# Autodesk Inventor assembly: high_joint
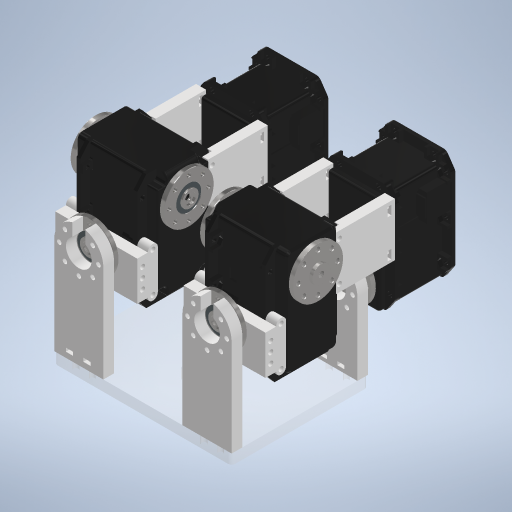
[picture p0: Inventor's stored thumbnail of the model, 512x512]
Saved by Autodesk Inventor 2024.3 (Build 283343000, 343)
## iProperties
Created: 2024-09-16
Part Number: high_joint
Document SubType Name: Assembly
Designer: USER
Author: USER
## Documents named in this file (10)
- C:\Users\USER\Desktop\로빛 예비인턴\(git)19기 이원준 격투로봇 설계파일\Lower_body\high_joint.iam
- C:\Users\USER\Desktop\로빛 예비인턴\(git)19기 이원준 격투로봇 설계파일\Lower_body\_pelvis.ipt
- C:\Users\USER\Desktop\로빛 예비인턴\(git)19기 이원준 격투로봇 설계파일\Lower_body\_thigh_adt_body.ipt
- C:\Users\USER\Desktop\로빛 예비인턴\(git)19기 이원준 격투로봇 설계파일\Lower_body\_foot_adt.ipt
- C:\Users\USER\Desktop\로빛 예비인턴\(git)19기 이원준 격투로봇 설계파일\Lower_body\_idle_adt.ipt
- C:\Users\USER\Desktop\로빛 예비인턴\(git)19기 이원준 격투로봇 설계파일\Lower_body\_adle_adt_2.ipt
- C:\Users\USER\Desktop\로빛 예비인턴\(git)19기 이원준 격투로봇 설계파일\아이들러\64아이들러.iam
- C:\Users\USER\Desktop\로빛 예비인턴\(git)19기 이원준 격투로봇 설계파일\motor\Motor_64_no_idle_ver.iam
- C:\Users\USER\Desktop\로빛 예비인턴\(git)19기 이원준 격투로봇 설계파일\motor\Motor_106.iam
- C:\Users\USER\Desktop\로빛 예비인턴\(git)19기 이원준 격투로봇 설계파일\Lower_body\_108-64_adt.ipt
## Components (21 placed, 9 different names)
1. _pelvis:1 — 플러쉬:1, 플러쉬:2, 삽입:1, 삽입:2, 각도:4, 삽입:3, 삽입:4, 각도:5, 각도:8, 삽입:5, 삽입:6, 삽입:7, 삽입:8
2. _thigh_adt_body:3 — 삽입:1, 삽입:2, 각도:7, 삽입:24, 각도:11, 각도:12, 삽입:38
3. _thigh_adt_body:4 — 각도:4, 삽입:3, 삽입:4, 각도:6, 삽입:23, 각도:10, 각도:13, 삽입:39
4. _foot_adt:1 — 각도:5, 각도:6, 삽입:5, 삽입:6, 삽입:25
5. _foot_adt:2 — 각도:7, 각도:8, 삽입:7, 삽입:8, 삽입:26
6. _idle_adt:3
7. _idle_adt:4 — 삽입:29, 삽입:30
8. _adle_adt_2:2 — 삽입:17
9. 64아이들러:1 [sub-assembly] — 삽입:17, 삽입:24, 삽입:38
10. _idle_adt:5 — 삽입:27, 삽입:28
11. _idle_adt:6
12. _adle_adt_2:3
13. 64아이들러:2 [sub-assembly] — 삽입:23, 삽입:39
14. Motor_64_no_idle_ver:1 [sub-assembly] — 삽입:26, 삽입:35, 삽입:36, 삽입:37, 각도:16
15. Motor_64_no_idle_ver:2 [sub-assembly] — 삽입:25, 삽입:31, 삽입:32, 삽입:33, 삽입:34
16. Motor_106:1 [sub-assembly] — 각도:11, 각도:12, 삽입:29, 삽입:30, 각도:16
17. Motor_106:2 [sub-assembly] — 각도:10, 각도:13, 삽입:27, 삽입:28, 각도:15
18. _108-64_adt:1 — 각도:14, 삽입:35, 삽입:36
19. _108-64_adt:2 — 각도:14, 삽입:37
20. _108-64_adt:3 — 삽입:33, 삽입:34
21. _108-64_adt:4 — 삽입:31, 삽입:32, 각도:15
## Relationships (49: Insert 35, Angle 12, Flush 2)
- 플러쉬:1 [Flush]: _pelvis:1
- 플러쉬:2 [Flush]: _pelvis:1
- 삽입:1 [Insert]: _pelvis:1 ↔ _thigh_adt_body:3
- 삽입:2 [Insert]: _pelvis:1 ↔ _thigh_adt_body:3
- 각도:4 [Angle] (0 deg): _pelvis:1 ↔ _thigh_adt_body:4
- 삽입:3 [Insert]: _pelvis:1 ↔ _thigh_adt_body:4
- 삽입:4 [Insert]: _pelvis:1 ↔ _thigh_adt_body:4
- 각도:5 [Angle] (0 deg): _pelvis:1 ↔ _foot_adt:1
- 각도:6 [Angle] (0 deg): _thigh_adt_body:4 ↔ _foot_adt:1
- 각도:7 [Angle] (0 deg): _thigh_adt_body:3 ↔ _foot_adt:2
- 각도:8 [Angle] (0 deg): _pelvis:1 ↔ _foot_adt:2
- 삽입:5 [Insert]: _pelvis:1 ↔ _foot_adt:1
- 삽입:6 [Insert]: _pelvis:1 ↔ _foot_adt:1
- 삽입:7 [Insert]: _pelvis:1 ↔ _foot_adt:2
- 삽입:8 [Insert]: _pelvis:1 ↔ _foot_adt:2
- [Insert]: _idle_adt:4 ↔ _adle_adt_2:2
- [Insert]: _idle_adt:4 ↔ _adle_adt_2:2
- [Insert]: _idle_adt:3 ↔ _adle_adt_2:2
- [Insert]: _idle_adt:3 ↔ _adle_adt_2:2
- 삽입:17 [Insert]: _adle_adt_2:2 ↔ 64아이들러:1
- [Insert]: _idle_adt:6 ↔ _adle_adt_2:3
- [Insert]: _idle_adt:6 ↔ _adle_adt_2:3
- [Insert]: _idle_adt:5 ↔ _adle_adt_2:3
- [Insert]: _idle_adt:5 ↔ _adle_adt_2:3
- [Insert]: _adle_adt_2:3 ↔ 64아이들러:2
- 삽입:23 [Insert]: _thigh_adt_body:4 ↔ 64아이들러:2
- 삽입:24 [Insert]: _thigh_adt_body:3 ↔ 64아이들러:1
- 삽입:25 [Insert]: _foot_adt:1 ↔ Motor_64_no_idle_ver:2
- 삽입:26 [Insert]: _foot_adt:2 ↔ Motor_64_no_idle_ver:1
- 각도:10 [Angle] (0 deg): _thigh_adt_body:4 ↔ Motor_106:2
- 각도:11 [Angle] (0 deg): _thigh_adt_body:3 ↔ Motor_106:1
- 각도:12 [Angle] (0 deg): _thigh_adt_body:3 ↔ Motor_106:1
- 각도:13 [Angle] (0 deg): _thigh_adt_body:4 ↔ Motor_106:2
- 각도:14 [Angle] (0 deg): _108-64_adt:1 ↔ _108-64_adt:2
- 삽입:27 [Insert]: _idle_adt:5 ↔ Motor_106:2
- 삽입:28 [Insert]: _idle_adt:5 ↔ Motor_106:2
- 삽입:29 [Insert]: _idle_adt:4 ↔ Motor_106:1
- 삽입:30 [Insert]: _idle_adt:4 ↔ Motor_106:1
- 삽입:31 [Insert]: Motor_64_no_idle_ver:2 ↔ _108-64_adt:4
- 삽입:32 [Insert]: Motor_64_no_idle_ver:2 ↔ _108-64_adt:4
- 각도:15 [Angle] (0 deg): Motor_106:2 ↔ _108-64_adt:4
- 삽입:33 [Insert]: Motor_64_no_idle_ver:2 ↔ _108-64_adt:3
- 삽입:34 [Insert]: Motor_64_no_idle_ver:2 ↔ _108-64_adt:3
- 삽입:35 [Insert]: Motor_64_no_idle_ver:1 ↔ _108-64_adt:1
- 삽입:36 [Insert]: Motor_64_no_idle_ver:1 ↔ _108-64_adt:1
- 삽입:37 [Insert]: Motor_64_no_idle_ver:1 ↔ _108-64_adt:2
- 각도:16 [Angle] (0 deg): Motor_64_no_idle_ver:1 ↔ Motor_106:1
- 삽입:38 [Insert]: _thigh_adt_body:3 ↔ 64아이들러:1
- 삽입:39 [Insert]: _thigh_adt_body:4 ↔ 64아이들러:2
## Named parameters: d26_d22 = 0 mm, d27_d23 = 0 mm, d28_d24 = 0 mm, d29_d25 = 0 mm, d32_d26_d22 = 0 mm, d33_d27_d23 = 0 mm, d34_d28_d24 = 0 mm, d35_d29_d25 = 0 mm, d36_d30 = 0 mm
